# Autodesk Inventor assembly: ASY PRS 1610 charging hatch_1200
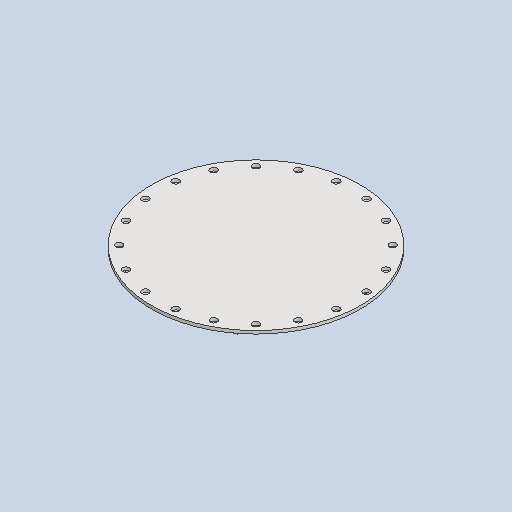
[picture p0: Inventor's stored thumbnail of the model, 512x512]
Saved by Autodesk Inventor 2026.2 (Build 302298000, 298)
## iProperties
Created: 2025-04-22
Part Number: ASY PRS 1610 charging hatch_1200
Document SubType Name: Assembly
Designer: admin
Mass: 9483.1 g
Surface Area: 9977.57 cm^2
Volume: 3616.18 cm^3
Density: 2.6224 g/cm^3
Author: user
## Documents named in this file (4)
- C:\Users\admin\Documents\Inventor\PRS-Purovsk\ASY PNS 1610 charging hatch_1200.iam
- C:\Users\admin\Documents\Inventor\PRS-Purovsk\SLM 1621 charging hatch D940_1200.ipt
- C:\Users\admin\Documents\Inventor\PRS-Purovsk\SLM 1611 hatch tube 500mm_1200.ipt
- C:\Users\admin\Documents\Inventor\PRS-Purovsk\SLM 1614 charging hatch reinf 500mm_1200.ipt
## Components (12 placed, 3 different names)
1. SLM 1621 charging hatch D940_1200:1 — Flush:1, Rigid:1
2. SLM 1611 hatch tube 500mm_1200:1 — Rigid:1
3. SLM 1614 charging hatch reinf 500mm_1200:1 — Mate:3, Mate:2, Flush:1, Mate:1
4. SLM 1614 charging hatch reinf 500mm_1200:2
5. SLM 1614 charging hatch reinf 500mm_1200:3
6. SLM 1614 charging hatch reinf 500mm_1200:4
7. SLM 1614 charging hatch reinf 500mm_1200:5
8. SLM 1614 charging hatch reinf 500mm_1200:6
9. SLM 1614 charging hatch reinf 500mm_1200:7
10. SLM 1614 charging hatch reinf 500mm_1200:8
11. SLM 1614 charging hatch reinf 500mm_1200:9
12. SLM 1614 charging hatch reinf 500mm_1200:10
## Component patterns: (10 elements, first: SLM 1614 charging hatch reinf 500mm_1200:1)
## Relationships (5: Mate 3, Flush 1, WeldJoint 1)
- Mate:3: SLM 1614 charging hatch reinf 500mm_1200:1
- Mate:2: SLM 1614 charging hatch reinf 500mm_1200:1
- Flush:1: SLM 1621 charging hatch D940_1200:1 ↔ SLM 1614 charging hatch reinf 500mm_1200:1
- Mate:1: SLM 1614 charging hatch reinf 500mm_1200:1
- Rigid:1 [WeldJoint]: SLM 1621 charging hatch D940_1200:1 ↔ SLM 1611 hatch tube 500mm_1200:1
